# Autodesk Inventor assembly: FlangeMountHousing
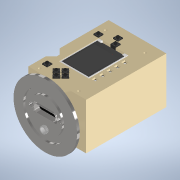
[picture p0: Inventor's stored thumbnail of the model, 180x180]
Saved by Autodesk Inventor 2022 (Build 260153070, 153G)
## iProperties
Created: 2021-12-02
Part Number: FlangeMountHousing
Document SubType Name: Assembly
Designer: elmar
Author: elmar
## iProperties of the stored document ST10U.ipt
Created: 2014-07-01
Part Number: ST10U
Material: Generic
Description: STEP AP214
Document SubType Name: Modeling
Designer: elmar
Density: 1 g/cm^3
Appearance: Default
Sending System: SolidWorks 2014
Preprocessor: SwSTEP 2.0
Title: ST10U.STEP
Revision Number: ANY
## Documents named in this file (7)
- D:\MyRepos\IRheating\3dModels\FlangeMountHousing.iam
- D:\MyRepos\IRheating\3dModels\KF50FeedThrough.ipt
- **D:\MyRepos\IRheating\3dModels\FlangeMountHousing.iam*LocalDocs*xAaaaaodaAaaaaaaaAaaaq3frIe*ST10U.ipt
- D:\MyRepos\IRheating\3dModels\A-HDS_26_LL-WP.ipt
- D:\MyRepos\IRheating\3dModels\PyBadge\PyBadge.iam
- D:\MyRepos\IRheating\3dModels\FeedthroughHousing.ipt
- D:\MyRepos\IRheating\3dModels\ST10U.STEP
## Components (5 placed, 5 different names)
1. KF50FeedThrough:1 — Insert:1, Insert:2, Angle:1, Flush:1, Flush:2, Mate:1, Mate:3
2. ST10U:1 — Insert:1
3. A-HDS_26_LL-WP:1 — Insert:2, Angle:1, Mate:2
4. PyBadge:1 [sub-assembly] — Mate:1, Mate:2, Mate:3, Flush:3, Flush:4, Flush:5, Flush:6
5. FeedthroughHousing:1 — Flush:1, Flush:2, Flush:3, Flush:4, Flush:5, Flush:6
## Relationships (12: Flush 6, Mate 3, Insert 2, Angle 1)
- Insert:1: KF50FeedThrough:1 ↔ ST10U:1
- Insert:2: KF50FeedThrough:1 ↔ A-HDS_26_LL-WP:1
- Angle:1 (0 deg): KF50FeedThrough:1 ↔ A-HDS_26_LL-WP:1
- Flush:1: KF50FeedThrough:1 ↔ FeedthroughHousing:1
- Flush:2: KF50FeedThrough:1 ↔ FeedthroughHousing:1
- Mate:1 (10 mm): KF50FeedThrough:1 ↔ PyBadge:1
- Mate:2 (8 mm): A-HDS_26_LL-WP:1 ↔ PyBadge:1
- Mate:3 (25 mm): KF50FeedThrough:1 ↔ PyBadge:1
- Flush:3: PyBadge:1 ↔ FeedthroughHousing:1
- Flush:4 (1 mm): PyBadge:1 ↔ FeedthroughHousing:1
- Flush:5 (5 mm): PyBadge:1 ↔ FeedthroughHousing:1
- Flush:6 (3 mm): PyBadge:1 ↔ FeedthroughHousing:1
